# Autodesk Inventor assembly: Frame Horizontals
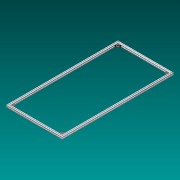
[picture p0: Inventor's stored thumbnail of the model, 180x180]
Saved by Autodesk Inventor 2016 (Build 200138000, 138)
## iProperties
Created: 2015-06-02
Part Number: Frame Horizontals
Document SubType Name: Assembly
Designer: Sawaiz Syed
Author: Sawaiz Syed
## Documents named in this file (5)
- C:\Users\Cosmic\Documents\Inventor\Black Box\Frame Horizontals.iam
- C:\Users\Admin\SkyDrive\Classes\Reaserch\Black Box\HFS5-2020.ipt
- C:\Users\Cosmic\Documents\Inventor\Black Box\HFS5-2020-1000.ipt
- C:\Users\Cosmic\Documents\Inventor\Black Box\HFS5-2020-460.ipt
- C:\Users\Cosmic\Documents\Inventor\Black Box\90 Barcket.iam
## Components (8 placed, 3 different names)
1. HFS5-2020-1000:1 — Flush:1, Flush:2, Flush:3, Flush:4, Mate:2, Flush:5, Mate:3, Flush:8, Flush:10, Mate:7, Mate:9
2. HFS5-2020-1000:2 — Flush:1, Flush:2, Mate:1, Flush:6, Mate:5, Mate:10
3. HFS5-2020-460:3 — Flush:3, Mate:2, Flush:5, Flush:9, Mate:8, Mate:11
4. HFS5-2020-460:4 — Flush:4, Mate:1, Flush:6, Mate:3, Flush:7, Mate:4, Mate:6
5. 90 Barcket:1 [sub-assembly] — Flush:7, Mate:4, Mate:5
6. 90 Barcket:2 [sub-assembly] — Flush:10, Mate:6, Mate:7
7. 90 Barcket:3 [sub-assembly] — Flush:9, Mate:10, Mate:11
8. 90 Barcket:4 [sub-assembly] — Flush:8, Mate:8, Mate:9
## Relationships (21: Mate 11, Flush 10)
- Flush:1: HFS5-2020-1000:1 ↔ HFS5-2020-1000:2
- Flush:2: HFS5-2020-1000:1 ↔ HFS5-2020-1000:2
- Flush:3: HFS5-2020-1000:1 ↔ HFS5-2020-460:3
- Flush:4: HFS5-2020-1000:1 ↔ HFS5-2020-460:4
- Mate:1: HFS5-2020-1000:2 ↔ HFS5-2020-460:4
- Mate:2: HFS5-2020-1000:1 ↔ HFS5-2020-460:3
- Flush:5: HFS5-2020-1000:1 ↔ HFS5-2020-460:3
- Flush:6: HFS5-2020-1000:2 ↔ HFS5-2020-460:4
- Mate:3: HFS5-2020-1000:1 ↔ HFS5-2020-460:4
- Flush:7: HFS5-2020-460:4 ↔ 90 Barcket:1
- Mate:4: HFS5-2020-460:4 ↔ 90 Barcket:1
- Mate:5: HFS5-2020-1000:2 ↔ 90 Barcket:1
- Flush:8: HFS5-2020-1000:1 ↔ 90 Barcket:4
- Flush:9: HFS5-2020-460:3 ↔ 90 Barcket:3
- Flush:10: HFS5-2020-1000:1 ↔ 90 Barcket:2
- Mate:6: HFS5-2020-460:4 ↔ 90 Barcket:2
- Mate:7: HFS5-2020-1000:1 ↔ 90 Barcket:2
- Mate:8: HFS5-2020-460:3 ↔ 90 Barcket:4
- Mate:9: HFS5-2020-1000:1 ↔ 90 Barcket:4
- Mate:10: HFS5-2020-1000:2 ↔ 90 Barcket:3
- Mate:11: HFS5-2020-460:3 ↔ 90 Barcket:3
